# Autodesk Inventor assembly: VersaWheel 2 sprockets for Drive in a Day 2013
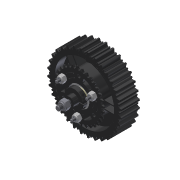
[picture p0: Inventor's stored thumbnail of the model, 180x180]
Saved by Autodesk Inventor 2013 (Build 170138000, 138)
## iProperties
Created: 2013-05-20
Part Number: VersaWheel 2 sprockets for Drive in a Day 2013
Document SubType Name: Assembly
Designer: Nemo
Author: Nemo
## Documents named in this file (11)
- H:\Nemo\Documents\Robotics\COTS Parts\Drive in a Day\VersaWheel 2 sprockets for Drive in a Day 2013.iam
- H:\Nemo\Documents\Robotics\Training Drive Base\Components\VexPro VersaWheel 4in.ipt
- H:\Nemo\Documents\Robotics\COTS Parts\Sprockets - VexPro #25\25 Sprocket 32T Vex.ipt
- H:\Nemo\Documents\Robotics\COTS Parts\Bearings - VexPro\Flanged Bearing - 0.5in Round ID x 1.125in OD.ipt
- H:\Nemo\Documents\Robotics\COTS Parts\Fasteners\8-32 locknut.ipt
- H:\Nemo\Documents\Robotics\COTS Parts\Fasteners\8-32 BHCS x2000.ipt
- H:\Nemo\Documents\Robotics\COTS Parts\Fasteners\500 Round Coupler.ipt
- H:\Nemo\Documents\Robotics\COTS Parts\Fasteners\500 Hex Spacer.ipt
- H:\Nemo\Documents\Robotics\COTS Parts\Drive in a Day\Tube Axle 2500 in.ipt
- H:\Nemo\Documents\Robotics\COTS Parts\Fasteners\14-20 locknut.ipt
- H:\Nemo\Documents\Robotics\COTS Parts\Fasteners\14-20 SHCS x3250.ipt
## Components (20 placed, 10 different names)
1. VexPro VersaWheel 4in:1
2. 25 Sprocket 32T Vex:1 — Insert:5
3. 25 Sprocket 32T Vex:2 — Insert:6
4. Flanged Bearing - 0.5in Round ID x 1.125in OD:1 — Insert:8
5. Flanged Bearing - 0.5in Round ID x 1.125in OD:2 — Mate:3, Insert:7
6. Tube Axle 2500 in:1 — Mate:3, Flush:1, Insert:13, Insert:14
7. 500 Round Coupler:2 — Insert:9
8. 500 Hex Spacer:1 — Insert:7, Insert:9
9. 500 Hex Spacer:2 — Insert:8, Insert:10
10. 500 Hex Spacer:3 — Insert:10, Insert:11
11. 500 Hex Spacer:4 — Insert:11, Insert:12
12. 500 Hex Spacer:5 — Insert:12, Flush:1
13. 14-20 locknut:1 — Insert:13
14. 14-20 SHCS x3250:1 — Insert:14
15. 8-32 locknut:1 — Insert:5
16. 8-32 BHCS x2000:1 — Insert:6
17. 8-32 locknut:2
18. 8-32 BHCS x2000:2
19. 8-32 locknut:3
20. 8-32 BHCS x2000:3
## Component patterns: (3 elements, first: 8-32 locknut:1 + 8-32 BHCS x2000:1)
## Relationships (18: Insert 14, Mate 3, Flush 1)
- [Insert]: VexPro VersaWheel 4in:1 ↔ Flanged Bearing - 0.5in Round ID x 1.125in OD:2
- [Insert]: VexPro VersaWheel 4in:1 ↔ Flanged Bearing - 0.5in Round ID x 1.125in OD:1
- [Insert]: VexPro VersaWheel 4in:1 ↔ 25 Sprocket 32T Vex:1
- [Mate]: VexPro VersaWheel 4in:1 ↔ 25 Sprocket 32T Vex:1
- [Insert]: VexPro VersaWheel 4in:1 ↔ 25 Sprocket 32T Vex:2
- [Mate]: VexPro VersaWheel 4in:1 ↔ 25 Sprocket 32T Vex:2
- Insert:5: 25 Sprocket 32T Vex:1 ↔ 8-32 locknut:1
- Insert:6: 25 Sprocket 32T Vex:2 ↔ 8-32 BHCS x2000:1
- Mate:3: Flanged Bearing - 0.5in Round ID x 1.125in OD:2 ↔ Tube Axle 2500 in:1
- Insert:7: Flanged Bearing - 0.5in Round ID x 1.125in OD:2 ↔ 500 Hex Spacer:1
- Insert:8: Flanged Bearing - 0.5in Round ID x 1.125in OD:1 ↔ 500 Hex Spacer:2
- Insert:9: 500 Round Coupler:2 ↔ 500 Hex Spacer:1
- Insert:10: 500 Hex Spacer:2 ↔ 500 Hex Spacer:3
- Insert:11: 500 Hex Spacer:3 ↔ 500 Hex Spacer:4
- Insert:12: 500 Hex Spacer:4 ↔ 500 Hex Spacer:5
- Flush:1: Tube Axle 2500 in:1 ↔ 500 Hex Spacer:5
- Insert:13 (3.175 mm): Tube Axle 2500 in:1 ↔ 14-20 locknut:1
- Insert:14 (3.175 mm): Tube Axle 2500 in:1 ↔ 14-20 SHCS x3250:1
